# Autodesk Inventor assembly: TITULEASA IOANA-ALEXANDRA_T7
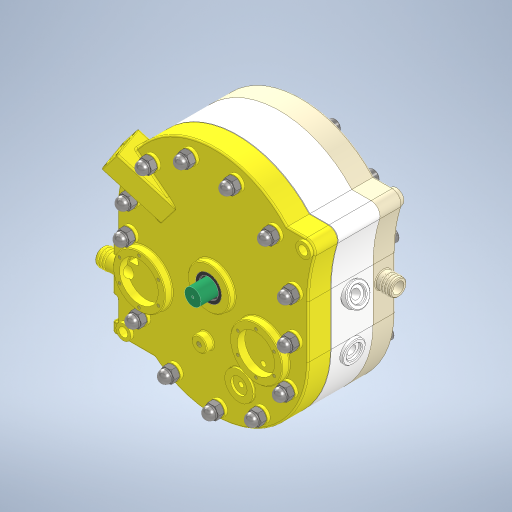
[picture p0: Inventor's stored thumbnail of the model, 512x512]
Saved by Autodesk Inventor 2024 (Build 280153000, 153)
## iProperties
Created: 2024-02-26
Part Number: TITULEASA IOANA-ALEXANDRA_T7
Document SubType Name: Assembly
Designer: mircea.oprea
YzzehuzbHJF: hkhfpsxbfrhyhshswbwfGwzijszahy5spJX689
eeniHffbFFJ: EyqsezmdhYDhmgwmezshygTDpVJsjhzuvpmjg
XdqhWwgibDJJ: EbpeyrbutfviVKuhrhb1
NuyvbdEFJ: PIHu4638
XgoomwwcdHEI: GJLsa2b65I
CobDFL: Wkj04z
UlrbdBDK: 3BpxepdqVnuwsvTbbsmlm
Author: mircea.oprea
## Documents named in this file (9)
- C:\Users\alexa\OneDrive\Documents\ANUL I\SEM 2\CAD\Tituleasa Ioana\TITULEASA IOANA-ALEXANDRA_T7.iam
- C:\Users\alexa\OneDrive\Documents\ANUL I\SEM 2\CAD\Fisiere auxiliare teme Inventor\Fisiere auxiliare teme Inventor\7 - Wankel\CapacSpate.ipt
- C:\Users\alexa\OneDrive\Documents\ANUL I\SEM 2\CAD\Fisiere auxiliare teme Inventor\Fisiere auxiliare teme Inventor\7 - Wankel\StatorWankel.ipt
- C:\Users\alexa\OneDrive\Documents\ANUL I\SEM 2\CAD\Fisiere auxiliare teme Inventor\Fisiere auxiliare teme Inventor\7 - Wankel\Arbore.ipt
- C:\Users\alexa\OneDrive\Documents\ANUL I\SEM 2\CAD\Tituleasa Ioana\SansRotor.iam
- C:\Users\alexa\OneDrive\Documents\ANUL I\SEM 2\CAD\Tituleasa Ioana\SansCapacFata.iam
- C:\Users\alexa\OneDrive\Documents\ANUL I\SEM 2\CAD\Tituleasa Ioana\Ans Suruburi Fixare.iam
- C:\Users\alexa\OneDrive\Documents\ANUL I\SEM 2\CAD\Tituleasa Ioana\Ans Piulite Fixare.iam
- C:\Users\alexa\OneDrive\Documents\Inventor\Content Center Files\R2024\en-US\ISO 6194 1  T 1\ISO 6194_1 - Type1 22 x 35 x 7.ipt
## Components (9 placed, 8 different names)
1. CapacSpate:2 — Mate:1, Mate:2, Angle:1, Mate:3, Mate:4, Mate:5, Mate:36
2. StatorWankel:1 — Mate:1, Mate:2, Angle:1, Angle Animation, Mate:7, Mate:9
3. Arbore:1 — Mate:3, Mate:4, Angle Animation, Mate:6, Angle:3, Rotation:1, Mate:8, Mate:37, Mate:39
4. SansRotor:1 [sub-assembly] — Mate:5, Mate:6, Angle:3, Rotation:1
5. SansCapacFata:1 [sub-assembly] — Mate:7, Mate:8, Mate:9, Mate:38
6. Ans Suruburi Fixare:1 [sub-assembly]
7. Ans Piulite Fixare:1 [sub-assembly]
8. ISO 6194/1 Type 1 Type1 22 x 35 x 7:1 — Mate:36, Mate:37
9. ISO 6194/1 Type 1 Type1 22 x 35 x 7:2 — Mate:38, Mate:39
## Relationships (32: Mate 27, Angle 3, RelateRotation 1, Insert 1)
- Mate:1: CapacSpate:2 ↔ StatorWankel:1
- Mate:2: CapacSpate:2 ↔ StatorWankel:1
- Angle:1 (0 deg): CapacSpate:2 ↔ StatorWankel:1
- Mate:3 (1 mm): CapacSpate:2 ↔ Arbore:1
- Mate:4: CapacSpate:2 ↔ Arbore:1
- Angle Animation (0 deg): StatorWankel:1 ↔ Arbore:1
- Mate:5: CapacSpate:2 ↔ SansRotor:1
- Mate:6: Arbore:1 ↔ SansRotor:1
- Angle:3 (0 deg): Arbore:1 ↔ SansRotor:1
- Rotation:1 [RelateRotation] (3 ul): Arbore:1 ↔ SansRotor:1
- Mate:7: StatorWankel:1 ↔ SansCapacFata:1
- Mate:8: Arbore:1 ↔ SansCapacFata:1
- Mate:9: StatorWankel:1 ↔ SansCapacFata:1
- [Insert]: SansCapacFata:1 ↔ Ans Suruburi Fixare:1
- [Mate]: Ans Suruburi Fixare:1 ↔ Ans Piulite Fixare:1
- [Mate]: CapacSpate:2 ↔ Ans Piulite Fixare:1
- [Mate]: CapacSpate:2 ↔ Ans Piulite Fixare:1
- [Mate]: CapacSpate:2 ↔ Ans Piulite Fixare:1
- [Mate]: CapacSpate:2 ↔ Ans Piulite Fixare:1
- [Mate]: CapacSpate:2 ↔ Ans Piulite Fixare:1
- [Mate]: CapacSpate:2 ↔ Ans Piulite Fixare:1
- [Mate]: CapacSpate:2 ↔ Ans Piulite Fixare:1
- [Mate]: CapacSpate:2 ↔ Ans Piulite Fixare:1
- [Mate]: CapacSpate:2 ↔ Ans Piulite Fixare:1
- [Mate]: CapacSpate:2 ↔ Ans Piulite Fixare:1
- [Mate]: CapacSpate:2 ↔ Ans Piulite Fixare:1
- [Mate]: CapacSpate:2 ↔ Ans Piulite Fixare:1
- [Mate]: CapacSpate:2 ↔ Ans Piulite Fixare:1
- Mate:36: CapacSpate:2 ↔ ISO 6194/1 Type 1 Type1 22 x 35 x 7:1
- Mate:37: Arbore:1 ↔ ISO 6194/1 Type 1 Type1 22 x 35 x 7:1
- Mate:38: SansCapacFata:1 ↔ ISO 6194/1 Type 1 Type1 22 x 35 x 7:2
- Mate:39: Arbore:1 ↔ ISO 6194/1 Type 1 Type1 22 x 35 x 7:2
